# Autodesk Inventor assembly: ballRampWithStepForBallRightSide
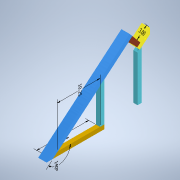
[picture p0: Inventor's stored thumbnail of the model, 180x180]
Saved by Autodesk Inventor 2020.2 (Build 242310000, 310)
## iProperties
Created: 2020-01-26
Part Number: ballRampWithStepForBallRightSide
Document SubType Name: Assembly
Designer: robst
Author: robst
## Documents named in this file (7)
- C:\git\CAD-Development\robSteele\2020CompetitionRobot\ballRampWithStepForBallRightSide.iam
- C:\git\CAD-Development\robSteele\2020CompetitionRobot\Aluminum1x1Base.ipt
- C:\git\CAD-Development\robSteele\2020CompetitionRobot\Aluminum1x2HypotLowerPortion.ipt
- C:\git\CAD-Development\robSteele\2020CompetitionRobot\Aluminum1x2Step.ipt
- C:\git\CAD-Development\robSteele\2020CompetitionRobot\Aluminum1x2HypotTop.ipt
- C:\git\CAD-Development\robSteele\2020CompetitionRobot\Aluminum1x1MiddleFront.ipt
- C:\git\CAD-Development\robSteele\2020CompetitionRobot\Aluminum1x1MiddleBack.ipt
## Components (6 placed, 6 different names)
1. Aluminum1x1Base:1 — Mate:4, Flush:7, Flush:8, Mate:5, Flush:9, Mate:6, Flush:10
2. Aluminum1x2HypotLowerPortion:1 — Mate:5, Flush:9, Mate:8, Flush:11, Flush:12
3. Aluminum1x2Step:1 — Mate:3, Flush:5, Flush:6, Mate:8, Flush:11, Flush:12
4. Aluminum1x2HypotTop:1 — Mate:3, Flush:5, Flush:6
5. Aluminum1x1MiddleFront:1 — Mate:4, Flush:7, Flush:8, Mate:7
6. Aluminum1x1MiddleBack:1 — Mate:6, Mate:7, Flush:10
## Relationships (14: Flush 8, Mate 6)
- Mate:3: Aluminum1x2Step:1 ↔ Aluminum1x2HypotTop:1
- Flush:5: Aluminum1x2Step:1 ↔ Aluminum1x2HypotTop:1
- Flush:6: Aluminum1x2Step:1 ↔ Aluminum1x2HypotTop:1
- Mate:4: Aluminum1x1Base:1 ↔ Aluminum1x1MiddleFront:1
- Flush:7: Aluminum1x1Base:1 ↔ Aluminum1x1MiddleFront:1
- Flush:8: Aluminum1x1Base:1 ↔ Aluminum1x1MiddleFront:1
- Mate:5: Aluminum1x1Base:1 ↔ Aluminum1x2HypotLowerPortion:1
- Flush:9: Aluminum1x1Base:1 ↔ Aluminum1x2HypotLowerPortion:1
- Mate:6: Aluminum1x1Base:1 ↔ Aluminum1x1MiddleBack:1
- Mate:7 (203.2 mm): Aluminum1x1MiddleFront:1 ↔ Aluminum1x1MiddleBack:1
- Flush:10: Aluminum1x1Base:1 ↔ Aluminum1x1MiddleBack:1
- Mate:8: Aluminum1x2HypotLowerPortion:1 ↔ Aluminum1x2Step:1
- Flush:11: Aluminum1x2HypotLowerPortion:1 ↔ Aluminum1x2Step:1
- Flush:12: Aluminum1x2HypotLowerPortion:1 ↔ Aluminum1x2Step:1
